# Autodesk Inventor assembly: Slider
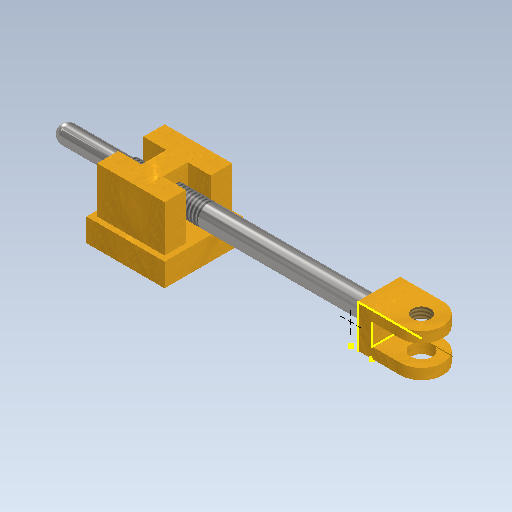
[picture p0: Inventor's stored thumbnail of the model, 512x512]
Saved by Autodesk Inventor 2020 (Build 240168000, 168)
## iProperties
Created: 2021-10-28
Part Number: Slider
Document SubType Name: Assembly
Designer: simon.erikssonwestl
Author: simon.erikssonwestl
## Documents named in this file (5)
- C:\Users\simon.erikssonwestl\Documents\Inventor\Ång\Assemblies\Slider.iam
- C:\Users\simon.erikssonwestl\Documents\Inventor\Ång\Part24.ipt
- C:\Users\simon.erikssonwestl\Documents\Inventor\Ång\Part23.ipt
- C:\Users\simon.erikssonwestl\Documents\Inventor\Ång\Part26.ipt
- C:\Users\simon.erikssonwestl\Documents\Inventor\Ång\Part27.ipt
## Components (4 placed, 4 different names)
1. Part24:1 — Mate:1, Mate:2, Angle:1
2. Part23:1 — Mate:1, Mate:2, Mate:3
3. Part26:1 — Mate:3, Angle:1, Mate:4, Mate:5, Flush:1
4. Part27:1 — Mate:4, Mate:5, Flush:1
## Relationships (7: Mate 5, Angle 1, Flush 1)
- Mate:1: Part24:1 ↔ Part23:1
- Mate:2: Part24:1 ↔ Part23:1
- Mate:3: Part23:1 ↔ Part26:1
- Angle:1 (0 deg): Part24:1 ↔ Part26:1
- Mate:4: Part26:1 ↔ Part27:1
- Mate:5: Part26:1 ↔ Part27:1
- Flush:1: Part26:1 ↔ Part27:1
